# Autodesk Inventor assembly: resevoir_mount
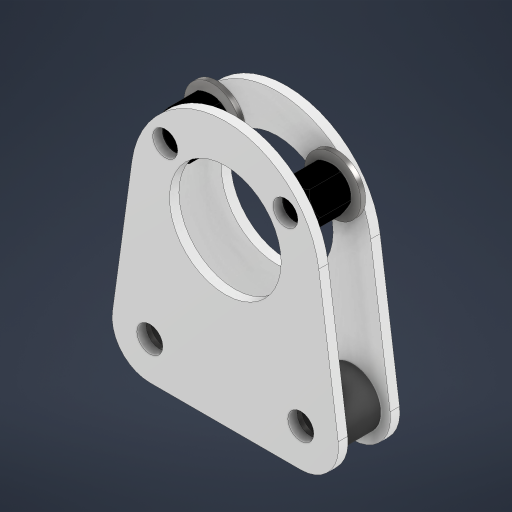
[picture p0: Inventor's stored thumbnail of the model, 512x512]
Saved by Autodesk Inventor 2024 (Build 280153000, 153)
## iProperties
Created: 2024-01-16
Part Number: resevoir_mount
Document SubType Name: Assembly
Designer: avere
Author: avere
## Documents named in this file (8)
- C:\Users\avere\Documents\rbp_cad\zoomba_v0.3\chassis\resevoir_mount.iam
- C:\Users\avere\Documents\rbp_cad\zoomba_v0.3\chassis\custom_parts\resevoir_mount.ipt
- C:\Users\avere\Documents\rbp_cad\VEX-CAD-Inventor-1.41\Structure\Standoff\Standoff .25.ipt
- C:\Users\avere\Documents\rbp_cad\VEX-CAD-Inventor-1.41\Structure\Standoff.ipt
- C:\Users\avere\Documents\rbp_cad\VEX-CAD-Inventor-1.41\Motion\Spacers\Spacer Nylon .375 OD\NSpacer .375 OD x .250.ipt
- C:\Users\avere\Documents\rbp_cad\VEX-CAD-Inventor-1.41\Motion\Spacers\Spacer Nylon .375 OD.ipt
- C:\Users\avere\Documents\rbp_cad\VEX-CAD-Inventor-1.41\Motion\Spacers\Washer Steel\SWasher .375 OD x .031250.ipt
- C:\Users\avere\Documents\rbp_cad\VEX-CAD-Inventor-1.41\Motion\Spacers\Washer Steel.ipt
## Components (10 placed, 4 different names)
1. resevoir_mount:1 — Mate:1, Insert:8, Insert:9
2. resevoir_mount:2 — Mate:1, Insert:10, Insert:11, Insert:12
3. Standoff .25:1 — Insert:12, Insert:14
4. Standoff .25:2 — Insert:11, Insert:13
5. NSpacer .375 OD x .250:1 — Insert:7, Insert:8
6. NSpacer .375 OD x .250:2 — Insert:6, Insert:9
7. SWasher .375 OD x .031250:1 — Insert:6
8. SWasher .375 OD x .031250:2 — Insert:7, Insert:10
9. SWasher .375 OD x .031250:3 — Insert:14
10. SWasher .375 OD x .031250:4 — Insert:13
## Relationships (10: Insert 9, Mate 1)
- Mate:1: resevoir_mount:1 ↔ resevoir_mount:2
- Insert:6: NSpacer .375 OD x .250:2 ↔ SWasher .375 OD x .031250:1
- Insert:7: NSpacer .375 OD x .250:1 ↔ SWasher .375 OD x .031250:2
- Insert:8: resevoir_mount:1 ↔ NSpacer .375 OD x .250:1
- Insert:9: resevoir_mount:1 ↔ NSpacer .375 OD x .250:2
- Insert:10: resevoir_mount:2 ↔ SWasher .375 OD x .031250:2
- Insert:11: resevoir_mount:2 ↔ Standoff .25:2
- Insert:12: resevoir_mount:2 ↔ Standoff .25:1
- Insert:13: Standoff .25:2 ↔ SWasher .375 OD x .031250:4
- Insert:14: Standoff .25:1 ↔ SWasher .375 OD x .031250:3
